# Autodesk Inventor assembly: s-assy-idler1
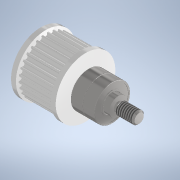
[picture p0: Inventor's stored thumbnail of the model, 180x180]
Saved by Autodesk Inventor 2022 (Build 260153000, 153)
## iProperties
Created: 2022-06-14
Part Number: s-assy-idler1
Document SubType Name: Assembly
Designer: yuto6
Author: yuto6
## Documents named in this file (4)
- C:\Users\yuto6\Documents\CAD\book-reader\s-assy-idler2.iam
- C:\Users\yuto6\Documents\CAD\book-reader\MR126ZZ.ipt
- C:\Users\yuto6\Documents\CAD\book-reader\MSB6-20.ipt
- C:\Users\yuto6\Documents\CAD\book-reader\base7.ipt
## Components (4 placed, 3 different names)
1. MR126ZZ:1 — メイト:4, メイト:6, メイト:8
2. MR126ZZ:2 — メイト:4, メイト:5
3. MSB6-20:1 — メイト:5, メイト:6, メイト:7, メイト:9
4. base7:1 — メイト:7, メイト:8, メイト:9
## Relationships (6: Mate 6)
- メイト:4 [Mate]: MR126ZZ:1 ↔ MR126ZZ:2
- メイト:5 [Mate]: MR126ZZ:2 ↔ MSB6-20:1
- メイト:6 [Mate]: MR126ZZ:1 ↔ MSB6-20:1
- メイト:7 [Mate]: MSB6-20:1 ↔ base7:1
- メイト:8 [Mate]: MR126ZZ:1 ↔ base7:1
- メイト:9 [Mate]: MSB6-20:1 ↔ base7:1
